# Autodesk Inventor assembly: STLassem
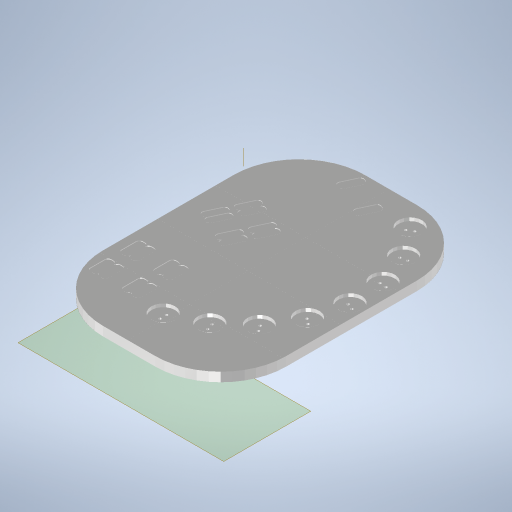
[picture p0: Inventor's stored thumbnail of the model, 512x512]
Saved by Autodesk Inventor 2024 (Build 280153000, 153)
## iProperties
Created: 2024-01-03
Part Number: STLassem
Document SubType Name: Assembly
Designer: Brian
Author: Brian
## Documents named in this file (28)
- C:\Users\brian\OneDrive\Documents\Inventor\drinkSilo\STLassem.iam
- C:\Users\brian\OneDrive\Documents\Inventor\drinkSilo\cutSTLs\B1.ipt
- C:\Users\brian\OneDrive\Documents\Inventor\drinkSilo\cutSTLs\B2.ipt
- C:\Users\brian\OneDrive\Documents\Inventor\drinkSilo\cutSTLs\B3.ipt
- C:\Users\brian\OneDrive\Documents\Inventor\drinkSilo\cutSTLs\B4.ipt
- C:\Users\brian\OneDrive\Documents\Inventor\drinkSilo\cutSTLs\B5.ipt
- C:\Users\brian\OneDrive\Documents\Inventor\drinkSilo\cutSTLs\B6.ipt
- C:\Users\brian\OneDrive\Documents\Inventor\drinkSilo\cutSTLs\B7.ipt
- C:\Users\brian\OneDrive\Documents\Inventor\drinkSilo\cutSTLs\B8.ipt
- C:\Users\brian\OneDrive\Documents\Inventor\drinkSilo\cutSTLs\P8.ipt
- C:\Users\brian\OneDrive\Documents\Inventor\drinkSilo\cutSTLs\P1.ipt
- C:\Users\brian\OneDrive\Documents\Inventor\drinkSilo\cutSTLs\P2.ipt
- C:\Users\brian\OneDrive\Documents\Inventor\drinkSilo\cutSTLs\P3.ipt
- C:\Users\brian\OneDrive\Documents\Inventor\drinkSilo\cutSTLs\P4.ipt
- C:\Users\brian\OneDrive\Documents\Inventor\drinkSilo\cutSTLs\P5.ipt
- C:\Users\brian\OneDrive\Documents\Inventor\drinkSilo\cutSTLs\P6.ipt
- C:\Users\brian\OneDrive\Documents\Inventor\drinkSilo\cutSTLs\P7.ipt
- C:\Users\brian\OneDrive\Documents\Inventor\drinkSilo\truckFront.ipt
- C:\Users\brian\OneDrive\Documents\Inventor\drinkSilo\truckBack.ipt
- C:\Users\brian\OneDrive\Documents\Inventor\drinkSilo\cutSTLs\Body2.ipt
- C:\Users\brian\OneDrive\Documents\Inventor\drinkSilo\cutSTLs\Body1.ipt
- C:\Users\brian\OneDrive\Documents\Inventor\drinkSilo\TrailerWheels.ipt
- C:\Users\brian\OneDrive\Documents\Inventor\drinkSilo\Micro Servo 9g.ipt
- C:\Users\brian\OneDrive\Documents\Inventor\drinkSilo\Part2.ipt
- C:\Users\brian\OneDrive\Documents\Inventor\drinkSilo\tube.ipt
- C:\Users\brian\OneDrive\Documents\Inventor\drinkSilo\glass.ipt
- C:\Users\brian\OneDrive\Documents\Inventor\drinkSilo\cutSTLs\Lid1.ipt
- C:\Users\brian\OneDrive\Documents\Inventor\drinkSilo\cutSTLs\Lid2.ipt
## Components (34 placed, 27 different names)
1. truckFront:1 — Mate:31, Mate:32, Mate:33
2. truckBack:1 — Mate:33, Mate:34, Mate:35, Mate:36, Insert:1
3. Body2:1 — Mate:37, Flush:19, Flush:20, Mate:38, Flush:21
4. Body1:2 — Mate:37, Flush:19, Flush:20, Insert:1, Angle:2, Mate:39, Flush:22, Flush:23, Flush:26, Mate:43, Flush:27
5. TrailerWheels:1 — Mate:38, Flush:21, Mate:40
6. Micro Servo 9g:1 — Mate:39, Flush:22, Flush:23, Rotational:1, Mate:41
7. Part2:1 — Rotational:1, Rigid:1
8. tube:1 — Rigid:1
9. glass:1 — Insert:2
10. glass:2 — Insert:3
11. glass:3 — Insert:4
12. glass:4 — Insert:5
13. glass:5 — Insert:7
14. glass:6 — Insert:8
15. glass:7 — Insert:9
16. glass:8 — Insert:6
17. Lid1:1 — Mate:42, Flush:24, Flush:25, Flush:26, Mate:43, Flush:27
18. Lid2:1 — Mate:42, Flush:24, Flush:25
19. B1:1 — Mate:29, Mate:18, Flush:14, Mate:19, Flush:15, Mate:22, Mate:23, Mate:27
20. B2:1 — Mate:17, Flush:13, Mate:18, Flush:14, Mate:23, Mate:24, Angle:1, Mate:30
21. B3:1 — Mate:15, Flush:12, Mate:16, Mate:17, Flush:13, Mate:24, Mate:28
22. B4:1 — Mate:13, Flush:11, Mate:14, Mate:15, Flush:12, Mate:16
23. B5:1 — Mate:13, Flush:11, Mate:14, Mate:26
24. B6:1 — Mate:21, Flush:17, Mate:26
25. B7:1 — Mate:20, Flush:16, Mate:21, Flush:17, Mate:25
26. B8:1 — Mate:19, Flush:15, Mate:20, Flush:16, Mate:22, Mate:25, Angle:2
27. P8:1 — Mate:8, Flush:6, Flush:7, Mate:12, Flush:9, Mate:30, Insert:2
28. P1:1 — Flush:1, Mate:1, Mate:2, Mate:3, Mate:4, Flush:2, Mate:31, Mate:32
29. P2:1 — Flush:1, Mate:1, Mate:2, Mate:5, Flush:3, Insert:7, Insert:8, Insert:9
30. P3:1 — Mate:3, Mate:4, Flush:2, Mate:6, Mate:10, Flush:8, Flush:18, Mate:34, Mate:35, Mate:36
31. P4:1 — Mate:5, Mate:6, Flush:3, Mate:7, Flush:4, Flush:5, Insert:6
32. P5:1 — Mate:10, Flush:8, Mate:11, Mate:29, Flush:18
33. P6:1 — Mate:7, Flush:4, Flush:5, Mate:8, Flush:6, Flush:7, Mate:28, Insert:3, Insert:4, Insert:5
34. P7:1 — Mate:11, Mate:12, Flush:9, Mate:40
## Relationships (81: Mate 42, Flush 26, Insert 9, Angle 2, RevoluteJoint 1, WeldJoint 1)
- Flush:1: P1:1 ↔ P2:1
- Mate:1: P1:1 ↔ P2:1
- Mate:2: P1:1 ↔ P2:1
- Mate:3: P1:1 ↔ P3:1
- Mate:4: P1:1 ↔ P3:1
- Flush:2: P1:1 ↔ P3:1
- Mate:5: P2:1 ↔ P4:1
- Mate:6: P3:1 ↔ P4:1
- Flush:3: P2:1 ↔ P4:1
- Mate:7: P4:1 ↔ P6:1
- Flush:4: P4:1 ↔ P6:1
- Flush:5: P4:1 ↔ P6:1
- Mate:8: P8:1 ↔ P6:1
- Flush:6: P8:1 ↔ P6:1
- Flush:7: P8:1 ↔ P6:1
- Mate:10: P3:1 ↔ P5:1
- Flush:8: P3:1 ↔ P5:1
- Mate:11: P5:1 ↔ P7:1
- Mate:12: P8:1 ↔ P7:1
- Flush:9: P8:1 ↔ P7:1
- Mate:29: B1:1 ↔ P5:1
- Mate:13: B4:1 ↔ B5:1
- Flush:11: B4:1 ↔ B5:1
- Mate:14: B4:1 ↔ B5:1
- Mate:15: B3:1 ↔ B4:1
- Flush:12: B3:1 ↔ B4:1
- Mate:16: B3:1 ↔ B4:1
- Mate:17: B2:1 ↔ B3:1
- Flush:13: B2:1 ↔ B3:1
- Mate:18: B1:1 ↔ B2:1
- Flush:14: B1:1 ↔ B2:1
- Mate:19: B1:1 ↔ B8:1
- Flush:15: B1:1 ↔ B8:1
- Mate:20: B7:1 ↔ B8:1
- Flush:16: B7:1 ↔ B8:1
- Mate:21: B6:1 ↔ B7:1
- Flush:17: B6:1 ↔ B7:1
- Mate:22: B1:1 ↔ B8:1
- Mate:23: B1:1 ↔ B2:1
- Mate:24: B2:1 ↔ B3:1
- Mate:25: B7:1 ↔ B8:1
- Mate:26: B5:1 ↔ B6:1
- Mate:27: B1:1
- Angle:1 (0 deg): B2:1
- Mate:28: B3:1 ↔ P6:1
- Flush:18: P3:1 ↔ P5:1
- Mate:30: B2:1 ↔ P8:1
- Mate:31 (17.78 mm): truckFront:1 ↔ P1:1
- Mate:32: truckFront:1 ↔ P1:1
- Mate:33: truckFront:1 ↔ truckBack:1
- Mate:34 (17.78 mm): truckBack:1 ↔ P3:1
- Mate:35: truckBack:1 ↔ P3:1
- Mate:36 (-15.24 mm): truckBack:1 ↔ P3:1
- Mate:37: Body2:1 ↔ Body1:2
- Flush:19: Body2:1 ↔ Body1:2
- Flush:20: Body2:1 ↔ Body1:2
- Insert:1: truckBack:1 ↔ Body1:2
- Angle:2 (0 deg): Body1:2 ↔ B8:1
- Mate:38: Body2:1 ↔ TrailerWheels:1
- Flush:21: Body2:1 ↔ TrailerWheels:1
- Mate:39: Body1:2 ↔ Micro Servo 9g:1
- Flush:22: Body1:2 ↔ Micro Servo 9g:1
- Flush:23: Body1:2 ↔ Micro Servo 9g:1
- Rotational:1 [RevoluteJoint]: Micro Servo 9g:1 ↔ Part2:1
- Rigid:1 [WeldJoint]: Part2:1 ↔ tube:1
- Mate:40: TrailerWheels:1 ↔ P7:1
- Insert:2: glass:1 ↔ P8:1
- Mate:41: Micro Servo 9g:1
- Insert:3: glass:2 ↔ P6:1
- Insert:4: glass:3 ↔ P6:1
- Insert:5: glass:4 ↔ P6:1
- Insert:6: glass:8 ↔ P4:1
- Insert:7: glass:5 ↔ P2:1
- Insert:8: glass:6 ↔ P2:1
- Insert:9: glass:7 ↔ P2:1
- Mate:42: Lid1:1 ↔ Lid2:1
- Flush:24: Lid1:1 ↔ Lid2:1
- Flush:25: Lid1:1 ↔ Lid2:1
- Flush:26: Body1:2 ↔ Lid1:1
- Mate:43: Body1:2 ↔ Lid1:1
- Flush:27: Body1:2 ↔ Lid1:1
